# Autodesk Inventor assembly: PS20030
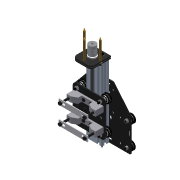
[picture p0: Inventor's stored thumbnail of the model, 180x180]
Saved by Autodesk Inventor 2014 (Build 180170000, 170)
## iProperties
Created: 2013-11-25
Part Number: PS20030
Document SubType Name: Assembly
Designer: Edward
Description: Complete Z-Axis Assembly
Author: Edward
Title: Complete Z-Axis Assembly
Subject: Shapeoko 2
## Documents named in this file (7)
- C:\Users\Edward\Documents\GitHub\Shapeoko_2\Autodesk_Inventor_Project\PS20030.iam
- C:\Users\Edward\Documents\GitHub\Shapeoko_2\Autodesk_Inventor_Project\PS20021.iam
- C:\Users\Edward\Documents\GitHub\Shapeoko_2\Autodesk_Inventor_Project\PS20028.iam
- C:\Users\Edward\Documents\GitHub\Shapeoko_2\Autodesk_Inventor_Project\PS20029.iam
- C:\Users\Edward\Documents\GitHub\Shapeoko_2\Autodesk_Inventor_Project\25287-02.ipt
- C:\Users\Edward\Documents\GitHub\Shapeoko_2\Autodesk_Inventor_Project\26016-01.ipt
- C:\Users\Edward\Documents\GitHub\Shapeoko_2\Autodesk_Inventor_Project\25286-01.ipt
## Components (15 placed, 6 different names)
1. PS20021:1 [sub-assembly] — Mate:1, Flush:1, Flush:2, Angle:1, Mate:3
2. PS20028:1 [sub-assembly] — Mate:1, Flush:1, Flush:2, Mate:2, Mate:4
3. PS20029:1 [sub-assembly] — Mate:2, Angle:1
4. 25287-02:1 — Mate:3
5. 26016-01:1 — Mate:4
6. 25286-01:1
7. 25287-02:2
8. 26016-01:2
9. 25286-01:2
10. 25287-02:3
11. 26016-01:3
12. 25286-01:3
13. 25287-02:4
14. 26016-01:4
15. 25286-01:4
## Component patterns: (4 elements, first: 25287-02:1 + 26016-01:1 + 25286-01:1)
## Relationships (9: Mate 4, Insert 2, Flush 2, Angle 1)
- [Insert]: 25287-02:1 ↔ 25286-01:1
- [Insert] (5.4163 mm): 25287-02:1 ↔ 26016-01:1
- Mate:1: PS20021:1 ↔ PS20028:1
- Flush:1: PS20021:1 ↔ PS20028:1
- Flush:2 (60 mm): PS20021:1 ↔ PS20028:1
- Mate:2: PS20028:1 ↔ PS20029:1
- Angle:1 (0 deg): PS20021:1 ↔ PS20029:1
- Mate:3: PS20021:1 ↔ 25287-02:1
- Mate:4 (1 mm): PS20028:1 ↔ 26016-01:1
## Named parameters: d159_d104 = 0 mm
